# Autodesk Inventor assembly: Bird_wing_assembly_V1
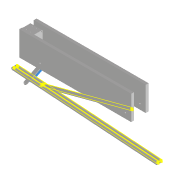
[picture p0: Inventor's stored thumbnail of the model, 180x180]
Saved by Autodesk Inventor 2022 (Build 260153000, 153)
## iProperties
Created: 2022-07-06
Part Number: Bird_wing_assembly_V1
Document SubType Name: Assembly
Designer: dell
Mass: 464.879 g
Surface Area: 1618.84 cm^2
Volume: 464.879 cm^3
Density: 1 g/cm^3
Author: dell
## Documents named in this file (8)
- D:\xxxx\Uni\Part IV\MECHENG_700\Part_IV_project_CAD\Bird_skeleton_prototypes\Wing_drone_V1\Bird_wing_V1\Bird_wing_assembly_V1.iam
- D:\xxxx\Uni\Part IV\MECHENG_700\Part_IV_project_CAD\Bird_skeleton_prototypes\Wing_drone_V1\Bird_wing_V1\Wing_base.ipt
- D:\xxxx\Uni\Part IV\MECHENG_700\Part_IV_project_CAD\Bird_skeleton_prototypes\Wing_drone_V1\Bird_wing_V1\Wing_arm_1.ipt
- D:\xxxx\Uni\Part IV\MECHENG_700\Part_IV_project_CAD\Bird_skeleton_prototypes\Wing_drone_V1\Bird_wing_V1\Wing_arm_2.ipt
- D:\xxxx\Uni\Part IV\MECHENG_700\Part_IV_project_CAD\Bird_skeleton_prototypes\Wing_drone_V1\Bird_wing_V1\Wing_arm_3.ipt
- D:\xxxx\Uni\Part IV\MECHENG_700\Part_IV_project_CAD\Bird_skeleton_prototypes\Wing_drone_V1\Bird_wing_V1\57545K764_Metal Worm Gear.ipt
- D:\xxxx\Uni\Part IV\MECHENG_700\Part_IV_project_CAD\Bird_skeleton_prototypes\Wing_drone_V1\Bird_wing_V1\Motor_assembly.iam
- D:\xxxx\Uni\Part IV\MECHENG_700\Part_IV_project_CAD\Bird_skeleton_prototypes\Wing_drone_V1\Bird_wing_V1\M3_washer.ipt
## Components (10 placed, 7 different names)
1. Wing_arm_1:1 — Mate:41, Mate:48, Mate:50, Mate:51, Mate:52
2. Wing_arm_1:2 — Mate:34, Mate:38, Mate:53
3. Wing_arm_2:1 — Flush:2, Mate:28, Mate:29
4. Wing_arm_2:2 — Flush:2
5. Wing_arm_3:1 — Mate:28, Mate:29, Mate:37
6. 57545K764_Metal Worm Gear:1 — Mate:34, Mate:38, Mate:50, Mate:51, Mate:52, Mate:53
7. Motor_assembly:5 [sub-assembly]
8. Wing_base:1 — Mate:37, Mate:41, Mate:42, Mate:43
9. M3_washer:1 — Mate:42, Mate:43, Mate:48
10. Wing_base:2
## Relationships (14: Mate 13, Flush 1)
- Flush:2: Wing_arm_2:1 ↔ Wing_arm_2:2
- Mate:28: Wing_arm_2:1 ↔ Wing_arm_3:1
- Mate:29: Wing_arm_2:1 ↔ Wing_arm_3:1
- Mate:34: Wing_arm_1:2 ↔ 57545K764_Metal Worm Gear:1
- Mate:37: Wing_arm_3:1 ↔ Wing_base:1
- Mate:38: Wing_arm_1:2 ↔ 57545K764_Metal Worm Gear:1
- Mate:41: Wing_arm_1:1 ↔ Wing_base:1
- Mate:42: Wing_base:1 ↔ M3_washer:1
- Mate:43: Wing_base:1 ↔ M3_washer:1
- Mate:48: Wing_arm_1:1 ↔ M3_washer:1
- Mate:50: Wing_arm_1:1 ↔ 57545K764_Metal Worm Gear:1
- Mate:51: Wing_arm_1:1 ↔ 57545K764_Metal Worm Gear:1
- Mate:52: Wing_arm_1:1 ↔ 57545K764_Metal Worm Gear:1
- Mate:53: Wing_arm_1:2 ↔ 57545K764_Metal Worm Gear:1
